# Autodesk Inventor assembly: IPT_TRACK_assembly
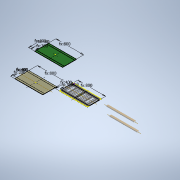
[picture p0: Inventor's stored thumbnail of the model, 180x180]
Saved by Autodesk Inventor 2021 (Build 250183000, 183)
## iProperties
Created: 2021-02-13
Part Number: IPT_TRACK_assembly
Document SubType Name: Assembly
Designer: phamv
Author: phamv
## Documents named in this file (5)
- C:\Users\phamv\OneDrive\UoA\2020 SUMMER\2020-srw-rc-car\CoilDesign\DEXTER_WORKSPACE\CAD stuff\Final_CAD\IPT_TRACK_assembly.iam
- C:\Users\phamv\OneDrive\UoA\2020 SUMMER\2020-srw-rc-car\CoilDesign\DEXTER_WORKSPACE\CAD stuff\Final_CAD\ferrite_layer_dex_1R1.ipt
- C:\Users\phamv\OneDrive\UoA\2020 SUMMER\2020-srw-rc-car\CoilDesign\DEXTER_WORKSPACE\CAD stuff\Final_CAD\coil_layer_1R1.ipt
- C:\Users\phamv\OneDrive\UoA\2020 SUMMER\2020-srw-rc-car\CoilDesign\DEXTER_WORKSPACE\CAD stuff\Final_CAD\track_surface_layer.ipt
- C:\Users\phamv\OneDrive\UoA\2020 SUMMER\2020-srw-rc-car\CoilDesign\DEXTER_WORKSPACE\CAD stuff\Final_CAD\track_walls.ipt
## Components (5 placed, 4 different names)
1. track_surface_layer:1 — Rigid:2, Rigid:3, Rigid:4
2. coil_layer_1R1:1 — Rigid:1, Rigid:2
3. ferrite_layer_dex_1R1:1 — Rigid:1
4. track_walls:1 — Rigid:3
5. track_walls:2 — Rigid:4
## Relationships (4: WeldJoint 4)
- Rigid:1 [WeldJoint]: coil_layer_1R1:1 ↔ ferrite_layer_dex_1R1:1
- Rigid:2 [WeldJoint]: track_surface_layer:1 ↔ coil_layer_1R1:1
- Rigid:3 [WeldJoint]: track_surface_layer:1 ↔ track_walls:1
- Rigid:4 [WeldJoint]: track_surface_layer:1 ↔ track_walls:2
